# Autodesk Inventor assembly: ASSEMBLY_Preamp
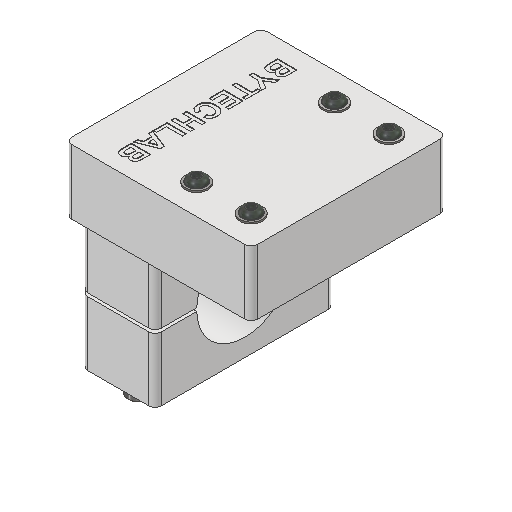
[picture p0: Inventor's stored thumbnail of the model, 512x512]
Saved by Autodesk Inventor 2026.1 (Build 301233000, 233)
## iProperties
Created: 2025-06-27
Part Number: ASSEMBLY_Preamp
Document SubType Name: Assembly
Designer: User
Author: User
## Documents named in this file (11)
- C:\Users\Andrzej\OneDrive\_DRIVE_SYNCH_FILES\__ BYTECHLAB PROJECTS\RF - Mostly 3D Printed Discone Antenna\MCAD\15_DISCONE_V4_KICAD\ASSEMBLY_PREAMP_REVA\ASSEMBLY_Preamp.iam
- C:\Users\Andrzej\OneDrive\_DRIVE_SYNCH_FILES\__ BYTECHLAB PROJECTS\RF - Mostly 3D Printed Discone Antenna\MCAD\15_DISCONE_V4_KICAD\ASSEMBLY_PREAMP_REVA\3DP_ASA_Preamp_Case_Bottom.ipt
- C:\Users\Andrzej\OneDrive\_DRIVE_SYNCH_FILES\__ BYTECHLAB PROJECTS\RF - Mostly 3D Printed Discone Antenna\MCAD\15_DISCONE_V4_KICAD\__COTS_PARTS\COTS_BOSSARD_1386867_M3_Insert.ipt
- C:\Users\Andrzej\OneDrive\_DRIVE_SYNCH_FILES\__ BYTECHLAB PROJECTS\RF - Mostly 3D Printed Discone Antenna\MCAD\15_DISCONE_V4_KICAD\ASSEMBLY_PREAMP_REVA\3DP_ASA_Preamp_Case_Top.ipt
- C:\Users\Andrzej\OneDrive\_DRIVE_SYNCH_FILES\__ BYTECHLAB PROJECTS\RF - Mostly 3D Printed Discone Antenna\MCAD\15_DISCONE_V4_KICAD\__CONTENT_CENTER_PARTS\en-US\DIN 125-1  A\DIN 125 - A 3,2.ipt
- C:\Users\Andrzej\OneDrive\_DRIVE_SYNCH_FILES\__ BYTECHLAB PROJECTS\RF - Mostly 3D Printed Discone Antenna\MCAD\15_DISCONE_V4_KICAD\__CONTENT_CENTER_PARTS\en-US\ISO 7380-1\ISO 7380-1 - M3 x 16.ipt
- C:\Users\Andrzej\OneDrive\_DRIVE_SYNCH_FILES\__ BYTECHLAB PROJECTS\RF - Mostly 3D Printed Discone Antenna\MCAD\15_DISCONE_V4_KICAD\ASSEMBLY_PREAMP_REVA\3DP_ASA_Preamp_Case_Clamp.ipt
- C:\Users\Andrzej\OneDrive\_DRIVE_SYNCH_FILES\__ BYTECHLAB PROJECTS\RF - Mostly 3D Printed Discone Antenna\MCAD\15_DISCONE_V4_KICAD\__CONTENT_CENTER_PARTS\en-US\DIN 125-1  A\DIN 125 - A 4,3.ipt
- C:\Users\Andrzej\OneDrive\_DRIVE_SYNCH_FILES\__ BYTECHLAB PROJECTS\RF - Mostly 3D Printed Discone Antenna\MCAD\15_DISCONE_V4_KICAD\__COTS_PARTS\COTS_GENERIC_DIN 912 - M4x50.ipt
- C:\Users\Andrzej\OneDrive\_DRIVE_SYNCH_FILES\__ BYTECHLAB PROJECTS\RF - Mostly 3D Printed Discone Antenna\MCAD\15_DISCONE_V4_KICAD\__CONTENT_CENTER_PARTS\en-US\DIN 934\DIN 934 - M4 x 0,7.ipt
- C:\Users\Andrzej\OneDrive\_DRIVE_SYNCH_FILES\__ BYTECHLAB PROJECTS\RF - Mostly 3D Printed Discone Antenna\MCAD\15_DISCONE_V4_KICAD\__KICAD_PCB_PARTS\3_PREAMP_PCB\ASSEMBLY_PREAMP_PCB.iam
## Components (22 placed, 10 different names)
1. 3DP_ASA_Preamp_Case_Bottom:1 — Mate:4, Mate:5, Mate:6, Mate:7, Flush:1, Flush:2, Flush:3, Flush:4, Mate:11, Flush:5, Flush:6, Mate:16, Mate:17, Angle:1, Angle:2, Mate:20
2. COTS_BOSSARD_1386867_M3_Insert:1 — Mate:4, Flush:3, Mate:24
3. COTS_BOSSARD_1386867_M3_Insert:2 — Mate:7, Flush:2, Mate:22, Mate:23
4. COTS_BOSSARD_1386867_M3_Insert:3 — Mate:5, Flush:4, Mate:21
5. COTS_BOSSARD_1386867_M3_Insert:4 — Mate:6, Flush:1
6. 3DP_ASA_Preamp_Case_Top:1 — Insert:1, Insert:2, Insert:3, Insert:4, Mate:25
7. DIN 125-1 A A 3,2:1 — Insert:1, Insert:5
8. DIN 125-1 A A 3,2:2 — Insert:2, Insert:8
9. DIN 125-1 A A 3,2:3 — Insert:3, Insert:7
10. DIN 125-1 A A 3,2:4 — Insert:4, Insert:6
11. ISO 7380-1 M3 x 16:1 — Insert:5, Mate:23
12. ISO 7380-1 M3 x 16:2 — Insert:6
13. ISO 7380-1 M3 x 16:3 — Insert:7, Mate:24
14. ISO 7380-1 M3 x 16:4 — Insert:8
15. 3DP_ASA_Preamp_Case_Clamp:1 — Mate:11, Flush:5, Flush:6, Insert:9, Insert:10, Mate:12, Mate:13
16. DIN 125-1 A A 4,3:1 — Insert:9, Mate:15
17. DIN 125-1 A A 4,3:2 — Insert:10, Mate:14
18. COTS_GENERIC_DIN 912 - M4x50:1 — Mate:12, Mate:15, Mate:19
19. COTS_GENERIC_DIN 912 - M4x50:2 — Mate:13, Mate:14, Mate:18
20. DIN 934 - replaced by DIN EN 24032/28673/28674 M4:1 — Mate:17, Mate:18, Angle:1
21. DIN 934 - replaced by DIN EN 24032/28673/28674 M4:2 — Mate:16, Mate:19, Angle:2
22. ASSEMBLY_PREAMP_PCB:1 [sub-assembly] — Mate:20, Mate:21, Mate:22, Mate:25
## Relationships (37: Mate 19, Insert 10, Flush 6, Angle 2)
- Mate:4: 3DP_ASA_Preamp_Case_Bottom:1 ↔ COTS_BOSSARD_1386867_M3_Insert:1
- Mate:5: 3DP_ASA_Preamp_Case_Bottom:1 ↔ COTS_BOSSARD_1386867_M3_Insert:3
- Mate:6: 3DP_ASA_Preamp_Case_Bottom:1 ↔ COTS_BOSSARD_1386867_M3_Insert:4
- Mate:7: 3DP_ASA_Preamp_Case_Bottom:1 ↔ COTS_BOSSARD_1386867_M3_Insert:2
- Flush:1: 3DP_ASA_Preamp_Case_Bottom:1 ↔ COTS_BOSSARD_1386867_M3_Insert:4
- Flush:2: 3DP_ASA_Preamp_Case_Bottom:1 ↔ COTS_BOSSARD_1386867_M3_Insert:2
- Flush:3: 3DP_ASA_Preamp_Case_Bottom:1 ↔ COTS_BOSSARD_1386867_M3_Insert:1
- Flush:4: 3DP_ASA_Preamp_Case_Bottom:1 ↔ COTS_BOSSARD_1386867_M3_Insert:3
- Insert:1: 3DP_ASA_Preamp_Case_Top:1 ↔ DIN 125-1 A A 3,2:1
- Insert:2: 3DP_ASA_Preamp_Case_Top:1 ↔ DIN 125-1 A A 3,2:2
- Insert:3: 3DP_ASA_Preamp_Case_Top:1 ↔ DIN 125-1 A A 3,2:3
- Insert:4: 3DP_ASA_Preamp_Case_Top:1 ↔ DIN 125-1 A A 3,2:4
- Insert:5: DIN 125-1 A A 3,2:1 ↔ ISO 7380-1 M3 x 16:1
- Insert:6: DIN 125-1 A A 3,2:4 ↔ ISO 7380-1 M3 x 16:2
- Insert:7: DIN 125-1 A A 3,2:3 ↔ ISO 7380-1 M3 x 16:3
- Insert:8: DIN 125-1 A A 3,2:2 ↔ ISO 7380-1 M3 x 16:4
- Mate:11 (1 mm): 3DP_ASA_Preamp_Case_Bottom:1 ↔ 3DP_ASA_Preamp_Case_Clamp:1
- Flush:5: 3DP_ASA_Preamp_Case_Bottom:1 ↔ 3DP_ASA_Preamp_Case_Clamp:1
- Flush:6: 3DP_ASA_Preamp_Case_Bottom:1 ↔ 3DP_ASA_Preamp_Case_Clamp:1
- Insert:9: 3DP_ASA_Preamp_Case_Clamp:1 ↔ DIN 125-1 A A 4,3:1
- Insert:10: 3DP_ASA_Preamp_Case_Clamp:1 ↔ DIN 125-1 A A 4,3:2
- Mate:12: 3DP_ASA_Preamp_Case_Clamp:1 ↔ COTS_GENERIC_DIN 912 - M4x50:1
- Mate:13: 3DP_ASA_Preamp_Case_Clamp:1 ↔ COTS_GENERIC_DIN 912 - M4x50:2
- Mate:14: DIN 125-1 A A 4,3:2 ↔ COTS_GENERIC_DIN 912 - M4x50:2
- Mate:15: DIN 125-1 A A 4,3:1 ↔ COTS_GENERIC_DIN 912 - M4x50:1
- Mate:16: 3DP_ASA_Preamp_Case_Bottom:1 ↔ DIN 934 - replaced by DIN EN 24032/28673/28674 M4:2
- Mate:17: 3DP_ASA_Preamp_Case_Bottom:1 ↔ DIN 934 - replaced by DIN EN 24032/28673/28674 M4:1
- Mate:18: COTS_GENERIC_DIN 912 - M4x50:2 ↔ DIN 934 - replaced by DIN EN 24032/28673/28674 M4:1
- Mate:19: COTS_GENERIC_DIN 912 - M4x50:1 ↔ DIN 934 - replaced by DIN EN 24032/28673/28674 M4:2
- Angle:1 (0 deg): 3DP_ASA_Preamp_Case_Bottom:1 ↔ DIN 934 - replaced by DIN EN 24032/28673/28674 M4:1
- Angle:2 (0 deg): 3DP_ASA_Preamp_Case_Bottom:1 ↔ DIN 934 - replaced by DIN EN 24032/28673/28674 M4:2
- Mate:20: 3DP_ASA_Preamp_Case_Bottom:1 ↔ ASSEMBLY_PREAMP_PCB:1
- Mate:21: COTS_BOSSARD_1386867_M3_Insert:3 ↔ ASSEMBLY_PREAMP_PCB:1
- Mate:22: COTS_BOSSARD_1386867_M3_Insert:2 ↔ ASSEMBLY_PREAMP_PCB:1
- Mate:23: COTS_BOSSARD_1386867_M3_Insert:2 ↔ ISO 7380-1 M3 x 16:1
- Mate:24: COTS_BOSSARD_1386867_M3_Insert:1 ↔ ISO 7380-1 M3 x 16:3
- Mate:25: 3DP_ASA_Preamp_Case_Top:1 ↔ ASSEMBLY_PREAMP_PCB:1
